# Autodesk Inventor assembly: OkiagariKoboshi
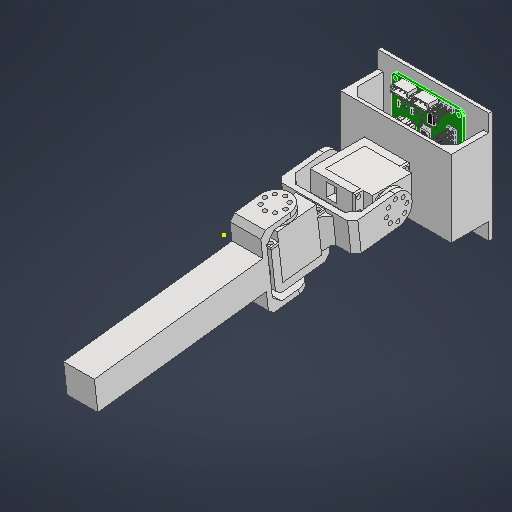
[picture p0: Inventor's stored thumbnail of the model, 512x512]
Saved by Autodesk Inventor 2026 (Build 300175050, 175E)
## iProperties
Created: 2026-07-07
Part Number: OkiagariKoboshi
Document SubType Name: Assembly
Designer: hanaj
Author: hanaj
## Documents named in this file (9)
- C:\Users\hanaj\OkiagariKoboshi_ws\CAD\OkiagariKoboshi.iam
- C:\Users\hanaj\OkiagariKoboshi_ws\CAD\STS3032.ipt
- C:\Users\hanaj\OkiagariKoboshi_ws\CAD\STS3032_Horn.ipt
- C:\Users\hanaj\OkiagariKoboshi_ws\CAD\Base.ipt
- C:\Users\hanaj\OkiagariKoboshi_ws\CAD\Arm1.ipt
- C:\Users\hanaj\OkiagariKoboshi_ws\CAD\Arm2.ipt
- C:\Users\hanaj\OkiagariKoboshi_ws\cad\Bus Servo Adapter (A)\Bus Servo Adapter (A)\Bus Servo Adapter (A).ipt
- C:\Users\hanaj\OkiagariKoboshi_ws\cad\M5Atom.ipt
- C:\Users\hanaj\OkiagariKoboshi_ws\cad\Battery.ipt
## Components (10 placed, 8 different names)
1. STS3032:1 — メイト:4, メイト:5, フラッシュ:1, 円柱状:1, メイト:9
2. STS3032_Horn:1 — 円柱状:1, メイト:9, メイト:10, メイト:11, メイト:12
3. Base:1 — メイト:4, メイト:5, フラッシュ:1, メイト:17, メイト:18, フラッシュ:3, メイト:19
4. Arm1:1 — メイト:7, メイト:8, フラッシュ:2, メイト:10, メイト:11, メイト:12
5. STS3032:2 — メイト:7, メイト:8, フラッシュ:2, 円柱状:2, メイト:13
6. STS3032_Horn:2 — 円柱状:2, メイト:13, メイト:14, メイト:15, メイト:16
7. Arm2:1 — メイト:14, メイト:15, メイト:16
8. Bus Servo Adapter (A):1 — メイト:18, フラッシュ:3, メイト:19
9. M5Atom:1
10. Battery:1 — メイト:17
## Relationships (20: Mate 15, Flush 3, CylindricalJoint 2)
- メイト:4 [Mate]: STS3032:1 ↔ Base:1
- メイト:5 [Mate]: STS3032:1 ↔ Base:1
- フラッシュ:1 [Flush]: STS3032:1 ↔ Base:1
- メイト:7 [Mate]: Arm1:1 ↔ STS3032:2
- メイト:8 [Mate]: Arm1:1 ↔ STS3032:2
- フラッシュ:2 [Flush]: Arm1:1 ↔ STS3032:2
- 円柱状:1 [CylindricalJoint]: STS3032:1 ↔ STS3032_Horn:1
- メイト:9 [Mate]: STS3032:1 ↔ STS3032_Horn:1
- メイト:10 [Mate]: STS3032_Horn:1 ↔ Arm1:1
- メイト:11 [Mate]: STS3032_Horn:1 ↔ Arm1:1
- メイト:12 [Mate]: STS3032_Horn:1 ↔ Arm1:1
- 円柱状:2 [CylindricalJoint]: STS3032:2 ↔ STS3032_Horn:2
- メイト:13 [Mate]: STS3032:2 ↔ STS3032_Horn:2
- メイト:14 [Mate]: STS3032_Horn:2 ↔ Arm2:1
- メイト:15 [Mate]: STS3032_Horn:2 ↔ Arm2:1
- メイト:16 [Mate]: STS3032_Horn:2 ↔ Arm2:1
- メイト:17 [Mate]: Base:1 ↔ Battery:1
- メイト:18 [Mate]: Base:1 ↔ Bus Servo Adapter (A):1
- フラッシュ:3 [Flush] (1 mm): Base:1 ↔ Bus Servo Adapter (A):1
- メイト:19 [Mate]: Base:1 ↔ Bus Servo Adapter (A):1
